# Autodesk Inventor assembly: Motor DC - MY1016Z
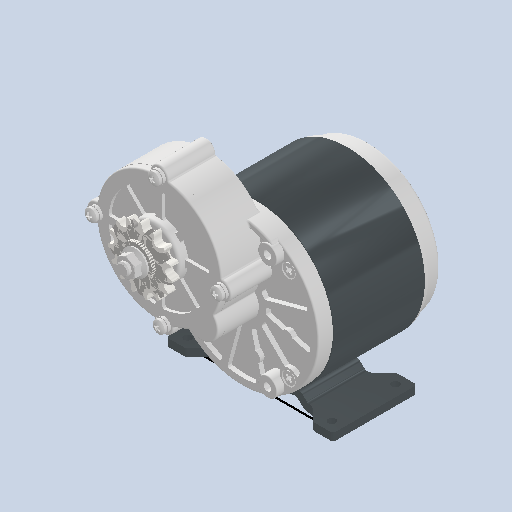
[picture p0: Inventor's stored thumbnail of the model, 512x512]
Saved by Autodesk Inventor 2023 (Build 270158000, 158)
## iProperties
Created: 2019-11-21
Part Number: Motor DC - MY1016Z
Description: STEP AP203
Document SubType Name: Assembly
Designer: sigit
Sending System: SolidWorks 2014
Preprocessor: SwSTEP 2.0
Title: Moteur DC - MY1016Z.STEP
Revision Number: ANY
## Documents named in this file (5)
- D:\Kuliah\SEMESTER 7\Robot Semprot\Design\REVISI2\Assembly\Motor DC - MY1016Z.iam
- D:\Kuliah\SEMESTER 7\Robot Semprot\Ref Design\motor dc\1016Z_stator.iam
- D:\Kuliah\SEMESTER 7\Robot Semprot\Ref Design\motor dc\1016Z_rotor.iam
- D:\Kuliah\SEMESTER 7\Robot Semprot\Ref Design\motor dc\1016Z_ensemble arbre de sortie.iam
- D:\Kuliah\SEMESTER 7\Robot Semprot\Design\REVISI2\Part\sprocket\Roller Chain Sprocket15.ipt
## Components (4 placed, 4 different names)
1. 1016Z_stator_1 [sub-assembly]
2. 1016Z_rotor_2 [sub-assembly]
3. 1016Z_ensemble arbre de sortie_3 [sub-assembly] — Rotational:1
4. Roller Chain Sprocket1:1 — Rotational:1
## Relationships (1: RevoluteJoint 1)
- Rotational:1 [RevoluteJoint]: 1016Z_ensemble arbre de sortie_3 ↔ Roller Chain Sprocket1:1
